# Autodesk Inventor assembly: ROBOT_ARM
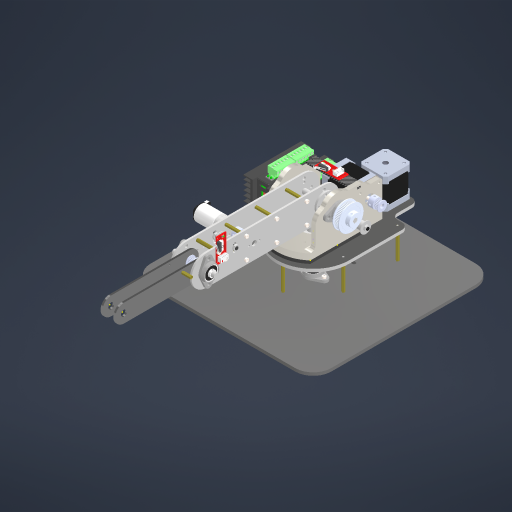
[picture p0: Inventor's stored thumbnail of the model, 512x512]
Saved by Autodesk Inventor 2023 (Build 270158000, 158)
## iProperties
Created: 2023-09-09
Part Number: ROBOT_ARM
Document SubType Name: Assembly
Designer: philo
Author: philo
## Documents named in this file (5)
- C:\Users\philo\OneDrive\Desktop\HK1-2024\TT ROBOT\02_3D_design_new\ROBOT_ARM.iam
- C:\Users\philo\OneDrive\Desktop\HK1-2024\TT ROBOT\02_3D_design_new\Base.iam
- C:\Users\philo\OneDrive\Desktop\HK1-2024\TT ROBOT\02_3D_design_new\Link2.iam
- C:\Users\philo\OneDrive\Desktop\HK1-2024\TT ROBOT\02_3D_design_new\Dexoay.iam
- C:\Users\philo\OneDrive\Desktop\HK1-2024\TT ROBOT\02_3D_design_new\Link3.iam
## Components (4 placed, 4 different names)
1. Base:1 [sub-assembly] — Mate:1, Flush:1, Angle:1
2. Link2:1 [sub-assembly] — Mate:2, Mate:3, Mate:4, Mate:5, Angle:2, Angle:3
3. Dexoay:1 [sub-assembly] — Mate:1, Flush:1, Mate:2, Mate:3, Angle:1, Angle:2
4. Link3:1 [sub-assembly] — Mate:4, Mate:5, Angle:3
## Relationships (9: Mate 5, Angle 3, Flush 1)
- Mate:1: Base:1 ↔ Dexoay:1
- Flush:1: Base:1 ↔ Dexoay:1
- Mate:2: Link2:1 ↔ Dexoay:1
- Mate:3 (15 mm): Link2:1 ↔ Dexoay:1
- Mate:4: Link2:1 ↔ Link3:1
- Mate:5: Link2:1 ↔ Link3:1
- Angle:1 (0 deg): Base:1 ↔ Dexoay:1
- Angle:2 (90 deg): Link2:1 ↔ Dexoay:1
- Angle:3 (0 deg): Link2:1 ↔ Link3:1
